# Autodesk Inventor assembly: The Final Chair (H)
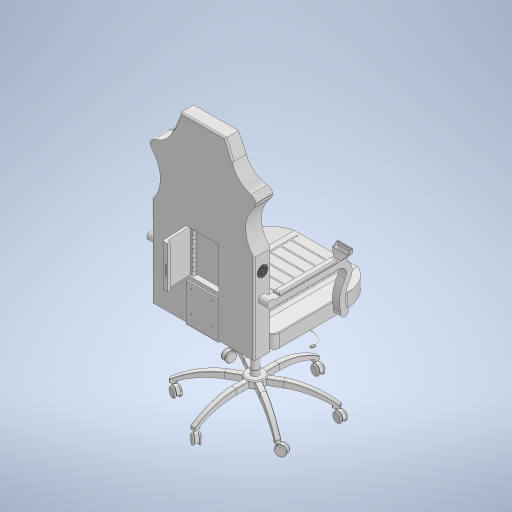
[picture p0: Inventor's stored thumbnail of the model, 512x512]
Saved by Autodesk Inventor 2023 (Build 270158030, 158C)
## iProperties
Created: 2023-03-03
Part Number: The Final Chair (H)
Document SubType Name: Assembly
Designer: mpino
Author: mpino
## Documents named in this file (13)
- C:\Users\mpino\Desktop\Cad\The Final Chair (H).iam
- C:\Users\mpino\Desktop\Cad\Base of chair (H).ipt
- C:\Users\mpino\Desktop\Cad\Full Wheel (H).iam
- C:\Users\mpino\Desktop\Cad\middle shaft.ipt
- C:\Users\mpino\Desktop\Cad\ChairBaseBracket.ipt
- C:\Users\mpino\Desktop\Cad\StandToBase (H).ipt
- C:\Users\mpino\Desktop\Cad\PivetRob(H).ipt
- C:\Users\mpino\Desktop\Cad\TheSeat(H).ipt
- C:\Users\mpino\Desktop\Cad\ConnectionBarcket(H).ipt
- C:\Users\mpino\Desktop\Cad\Back of Chair(H).ipt
- C:\Users\mpino\Desktop\Cad\PhoneSafeDoor(H).ipt
- C:\Users\mpino\Desktop\Cad\Speaker(H).ipt
- C:\Users\mpino\Desktop\Cad\Height adjust(H).ipt
## Components (18 placed, 12 different names)
1. Base of chair (H):1 — Mate:1, Mate:2, Mate:3, Mate:4, Mate:5, Mate:6, Mate:7, Mate:8, Mate:9, Mate:10, Mate:11, Mate:12, Mate:13, Mate:14
2. Full Wheel (H):1 [sub-assembly] — Mate:4, Mate:8
3. Full Wheel (H):2 [sub-assembly] — Mate:3, Mate:9
4. Full Wheel (H):3 [sub-assembly] — Mate:2, Mate:10
5. Full Wheel (H):4 [sub-assembly] — Mate:5, Mate:7
6. Full Wheel (H):5 [sub-assembly] — Mate:6, Mate:12
7. Full Wheel (H):6 [sub-assembly] — Mate:1, Mate:11
8. middle shaft:1 — Mate:13, Mate:14, Mate:15, Mate:16
9. ChairBaseBracket:1 — Mate:18, Mate:19, Mate:20, Mate:21, Mate:22, Mate:24, Mate:28, Mate:40
10. StandToBase (H):1 — Mate:15, Mate:16, Mate:18, Mate:19, Mate:29, Mate:39
11. PivetRob(H):1 — Mate:20, Mate:21, Mate:29
12. TheSeat(H):1 — Mate:22, Mate:24, Mate:25, Mate:26, Mate:27, Mate:28
13. ConnectionBarcket(H):1 — Mate:25, Mate:26, Mate:27, Mate:30, Mate:31, Mate:32
14. Back of Chair(H):1 — Mate:30, Mate:31, Mate:32, Mate:33, Mate:34, Mate:35, Mate:36, Mate:37, Mate:38
15. PhoneSafeDoor(H):1 — Mate:33, Mate:34
16. Speaker(H):1 — Mate:37, Mate:38
17. Speaker(H):2 — Mate:35, Mate:36
18. Height adjust(H):1 — Mate:39, Mate:40
## Relationships (38: Mate 38)
- Mate:1: Base of chair (H):1 ↔ Full Wheel (H):6
- Mate:2: Base of chair (H):1 ↔ Full Wheel (H):3
- Mate:3: Base of chair (H):1 ↔ Full Wheel (H):2
- Mate:4: Base of chair (H):1 ↔ Full Wheel (H):1
- Mate:5: Base of chair (H):1 ↔ Full Wheel (H):4
- Mate:6: Base of chair (H):1 ↔ Full Wheel (H):5
- Mate:7: Base of chair (H):1 ↔ Full Wheel (H):4
- Mate:8: Base of chair (H):1 ↔ Full Wheel (H):1
- Mate:9: Base of chair (H):1 ↔ Full Wheel (H):2
- Mate:10: Base of chair (H):1 ↔ Full Wheel (H):3
- Mate:11: Base of chair (H):1 ↔ Full Wheel (H):6
- Mate:12: Base of chair (H):1 ↔ Full Wheel (H):5
- Mate:13: Base of chair (H):1 ↔ middle shaft:1
- Mate:14: Base of chair (H):1 ↔ middle shaft:1
- Mate:15: middle shaft:1 ↔ StandToBase (H):1
- Mate:16: middle shaft:1 ↔ StandToBase (H):1
- Mate:18: ChairBaseBracket:1 ↔ StandToBase (H):1
- Mate:19: ChairBaseBracket:1 ↔ StandToBase (H):1
- Mate:20: ChairBaseBracket:1 ↔ PivetRob(H):1
- Mate:21: ChairBaseBracket:1 ↔ PivetRob(H):1
- Mate:22: ChairBaseBracket:1 ↔ TheSeat(H):1
- Mate:24: ChairBaseBracket:1 ↔ TheSeat(H):1
- Mate:25: TheSeat(H):1 ↔ ConnectionBarcket(H):1
- Mate:26: TheSeat(H):1 ↔ ConnectionBarcket(H):1
- Mate:27: TheSeat(H):1 ↔ ConnectionBarcket(H):1
- Mate:28: ChairBaseBracket:1 ↔ TheSeat(H):1
- Mate:29: StandToBase (H):1 ↔ PivetRob(H):1
- Mate:30: ConnectionBarcket(H):1 ↔ Back of Chair(H):1
- Mate:31: ConnectionBarcket(H):1 ↔ Back of Chair(H):1
- Mate:32: ConnectionBarcket(H):1 ↔ Back of Chair(H):1
- Mate:33: Back of Chair(H):1 ↔ PhoneSafeDoor(H):1
- Mate:34: Back of Chair(H):1 ↔ PhoneSafeDoor(H):1
- Mate:35: Back of Chair(H):1 ↔ Speaker(H):2
- Mate:36: Back of Chair(H):1 ↔ Speaker(H):2
- Mate:37: Back of Chair(H):1 ↔ Speaker(H):1
- Mate:38: Back of Chair(H):1 ↔ Speaker(H):1
- Mate:39: StandToBase (H):1 ↔ Height adjust(H):1
- Mate:40: ChairBaseBracket:1 ↔ Height adjust(H):1
